# Autodesk Inventor assembly: Assy_all
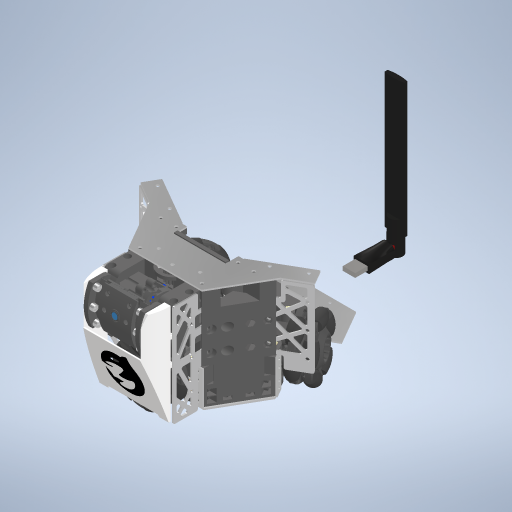
[picture p0: Inventor's stored thumbnail of the model, 512x512]
Saved by Autodesk Inventor 2024.1 (Build 281209000, 209)
## iProperties
Created: 2025-03-04
Part Number: Assy_all
Document SubType Name: Assembly
Designer: hibik
Author: hibik
## Documents named in this file (4)
- C:\Users\hibik\Documents\Robomech\RESCUE\ORCA\hard\Assy_all.iam
- C:\Users\hibik\Documents\Robomech\RESCUE\ORCA\hard\Assy_cam_connection.iam
- C:\Users\hibik\Documents\Robomech\RESCUE\ORCA\hard\std_parts\Buffalo_Wl-U2-433DHP.ipt
- C:\Users\hibik\Documents\Robomech\RESCUE\ORCA\hard\cover\cover_front.ipt
## Components (3 placed, 3 different names)
1. Assy_cam_connection:1 [sub-assembly] — 挿入:8, 角度:2
2. Buffalo_Wl-U2-433DHP:1
3. cover_front:1 — 挿入:8, 角度:2
## Relationships (2: Insert 1, Angle 1)
- 挿入:8 [Insert]: Assy_cam_connection:1 ↔ cover_front:1
- 角度:2 [Angle] (0 deg): Assy_cam_connection:1 ↔ cover_front:1
